# Autodesk Inventor assembly: zlozenie_na_strzykawke
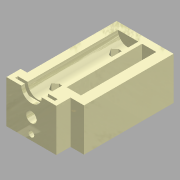
[picture p0: Inventor's stored thumbnail of the model, 180x180]
Saved by Autodesk Inventor 2021 (Build 250183000, 183)
## iProperties
Created: 2022-05-24
Part Number: zlozenie_na_strzykawke
Document SubType Name: Assembly
Designer: agnpi
Author: agnpi
## Documents named in this file (3)
- D:\users\agnpi\Desktop\lekcje\SEMESTR VII\Inventor video\Zlozenie inne kolory\zlozenie_na_strzykawke_.iam
- D:\users\agnpi\Desktop\lekcje\SEMESTR VII\Inventor video\Zlozenie inne kolory\uchwyt_strzykawka_dol_.ipt
- D:\users\agnpi\Desktop\lekcje\SEMESTR VII\Inventor video\Zlozenie inne kolory\uchwyt_strzykawka_srodek_proba_zapisania_.ipt
## Components (2 placed, 2 different names)
1. uchwyt_strzykawka_dol_:1
2. uchwyt_strzykawka_srodek_proba_zapisania_:1
## Relationships (5: Mate 5)
- [Mate]: uchwyt_strzykawka_dol_:1 ↔ uchwyt_strzykawka_srodek_proba_zapisania_:1
- [Mate]: uchwyt_strzykawka_dol_:1 ↔ uchwyt_strzykawka_srodek_proba_zapisania_:1
- [Mate]: uchwyt_strzykawka_dol_:1 ↔ uchwyt_strzykawka_srodek_proba_zapisania_:1
- [Mate]: uchwyt_strzykawka_dol_:1 ↔ uchwyt_strzykawka_srodek_proba_zapisania_:1
- [Mate]: uchwyt_strzykawka_dol_:1 ↔ uchwyt_strzykawka_srodek_proba_zapisania_:1
